# Autodesk Inventor assembly: 整车
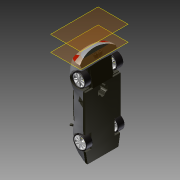
[picture p0: Inventor's stored thumbnail of the model, 180x180]
Saved by Autodesk Inventor 2012 (Build 160160000, 160)
## iProperties
Created: 2012-04-14
Part Number: 整车
Document SubType Name: Assembly
Designer: dell
Mass: 5.39099e+06 g
Surface Area: 432303 cm^2
Volume: 5.39099e+06 cm^3
Density: 1 g/cm^3
Author: dell
## Documents named in this file (7)
- F:\跑车\兰博基尼\整车.iam
- F:\跑车\兰博基尼\车身实体.ipt
- F:\跑车\兰博基尼\车灯.ipt
- F:\跑车\兰博基尼\前行李舱盖.ipt
- F:\跑车\兰博基尼\右视图.ipt
- F:\毕业设计\FEA\轮毂.ipt
- F:\毕业设计\FEA\轮胎.ipt
## Components (12 placed, 6 different names)
1. 车身实体:1 — 配合:1, 配合:2, 配合:3, 配合:4, 配合:5, 相切:1, 配合:6, 配合:7, 配合:9, 配合:10, 配合:11, 配合:12, 配合:13, 配合:14
2. 车灯:1 — 配合:1, 配合:2, 配合:3
3. 前行李舱盖:1 — 配合:4, 配合:5, 相切:1
4. 右视图:1 — 表面齐平:2
5. 轮毂:1 — 配合:6, 配合:9, 配合:16, 表面齐平:6
6. 轮毂:2 — 配合:7, 配合:13, 配合:15, 表面齐平:3
7. 轮毂:3 — 配合:11, 配合:12, 配合:17, 表面齐平:5
8. 轮毂:4 — 配合:10, 配合:14, 配合:18, 表面齐平:4
9. 轮胎:1 — 配合:15, 表面齐平:3
10. 轮胎:2 — 配合:17, 表面齐平:5
11. 轮胎:3 — 配合:16, 表面齐平:6
12. 轮胎:4 — 配合:18, 表面齐平:4
## Relationships (24: Mate 17, Flush 6, Tangent 1)
- 配合:1 [Mate]: 车身实体:1 ↔ 车灯:1
- 配合:2 [Mate]: 车身实体:1 ↔ 车灯:1
- 配合:3 [Mate]: 车身实体:1 ↔ 车灯:1
- 配合:4 [Mate]: 车身实体:1 ↔ 前行李舱盖:1
- 配合:5 [Mate]: 车身实体:1 ↔ 前行李舱盖:1
- 表面齐平:1 [Flush] (2000 mm)
- 表面齐平:2 [Flush]: 右视图:1
- 相切:1 [Tangent]: 车身实体:1 ↔ 前行李舱盖:1
- 配合:6 [Mate]: 车身实体:1 ↔ 轮毂:1
- 配合:7 [Mate]: 车身实体:1 ↔ 轮毂:2
- 配合:9 [Mate]: 车身实体:1 ↔ 轮毂:1
- 配合:10 [Mate]: 车身实体:1 ↔ 轮毂:4
- 配合:11 [Mate]: 车身实体:1 ↔ 轮毂:3
- 配合:12 [Mate]: 车身实体:1 ↔ 轮毂:3
- 配合:13 [Mate]: 车身实体:1 ↔ 轮毂:2
- 配合:14 [Mate]: 车身实体:1 ↔ 轮毂:4
- 配合:15 [Mate]: 轮毂:2 ↔ 轮胎:1
- 表面齐平:3 [Flush]: 轮毂:2 ↔ 轮胎:1
- 配合:16 [Mate]: 轮毂:1 ↔ 轮胎:3
- 配合:17 [Mate]: 轮毂:3 ↔ 轮胎:2
- 配合:18 [Mate]: 轮毂:4 ↔ 轮胎:4
- 表面齐平:4 [Flush]: 轮毂:4 ↔ 轮胎:4
- 表面齐平:5 [Flush]: 轮毂:3 ↔ 轮胎:2
- 表面齐平:6 [Flush]: 轮毂:1 ↔ 轮胎:3
